# Autodesk Inventor assembly: FarmBot
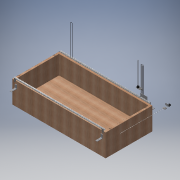
[picture p0: Inventor's stored thumbnail of the model, 180x180]
Saved by Autodesk Inventor 2017 (Build 210142000, 142)
## iProperties
Created: 2016-12-12
Part Number: FarmBot
Document SubType Name: Assembly
Designer: umr
Author: umr
## Documents named in this file (6)
- D:\SeniorProject\Models2\FarmBot.iam
- D:\SeniorProject\Models2\BedAssembly\BedAseembly.iam
- D:\SeniorProject\Models2\Case\Case.iam
- D:\SeniorProject\Models2\LED Structure\LED Structure Assembly.iam
- D:\SeniorProject\Models2\Gantry\GantryDown.iam
- D:\SeniorProject\Models2\BeltMain.ipt
## Components (5 placed, 5 different names)
1. BedAseembly:2 [sub-assembly] — Mate:10, Mate:11, Mate:12, Mate:13, Mate:14, Mate:15, Mate:16, Mate:18, Flush:1, Mate:19, Mate:20
2. Case:1 [sub-assembly] — Mate:10, Mate:11, Mate:12, Mate:13
3. LED Structure Assembly:1 [sub-assembly] — Mate:14, Mate:15, Mate:16
4. GantryDown:1 [sub-assembly] — Mate:18, Flush:1, Tangent:1
5. BeltMain:1 — Mate:19, Mate:20, Tangent:1
## Relationships (12: Mate 10, Flush 1, Tangent 1)
- Mate:10: BedAseembly:2 ↔ Case:1
- Mate:11: BedAseembly:2 ↔ Case:1
- Mate:12: BedAseembly:2 ↔ Case:1
- Mate:13: BedAseembly:2 ↔ Case:1
- Mate:14: BedAseembly:2 ↔ LED Structure Assembly:1
- Mate:15: BedAseembly:2 ↔ LED Structure Assembly:1
- Mate:16: BedAseembly:2 ↔ LED Structure Assembly:1
- Mate:18: BedAseembly:2 ↔ GantryDown:1
- Flush:1 (100 mm): BedAseembly:2 ↔ GantryDown:1
- Mate:19: BedAseembly:2 ↔ BeltMain:1
- Mate:20 (3 mm): BedAseembly:2 ↔ BeltMain:1
- Tangent:1: GantryDown:1 ↔ BeltMain:1
